# Autodesk Inventor assembly: Right Rear Wheel with hub
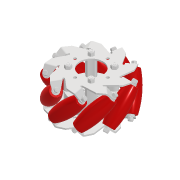
[picture p0: Inventor's stored thumbnail of the model, 180x180]
Saved by Autodesk Inventor 2020 (Build 240168000, 168)
## iProperties
Created: 2020-02-22
Part Number: Right Rear Wheel with hub
Document SubType Name: Assembly
Designer: ball
Author: ball
## Documents named in this file (5)
- C:\FTC\FTC8863CAD\2019 Robot\Mecanum Drive Train Metal\Right Rear Wheel with hub.iam
- C:\FTC\FTC8863CAD\GoBilda\1310 Parts\1310-0016-4008 assembly.ipt
- C:\FTC\FTC8863CAD\StepLibraries\Screws\M4 x 22 SOCKET HEAD CAP SCREW.ipt
- C:\FTC\FTC8863CAD\StepLibraries\Washers\M4 FLAT WASHER.ipt
- C:\FTC\FTC8863CAD\GoBilda\3213 Parts\3606-0000-0100 assembly.iam
## Components (10 placed, 4 different names)
1. 3606-0000-0100 assembly:1 [sub-assembly] — Mate:1, Mate:2, Mate:3, Mate:12, Mate:13, Mate:14, Mate:15, Mate:18, Mate:19, Mate:22, Mate:23
2. 1310-0016-4008 assembly:1 — Mate:1, Mate:2, Mate:3
3. M4 x 22 SOCKET HEAD CAP SCREW:1 — Mate:13
4. M4 FLAT WASHER:1 — Mate:12
5. M4 x 22 SOCKET HEAD CAP SCREW:3 — Mate:19
6. M4 FLAT WASHER:3 — Mate:18
7. M4 x 22 SOCKET HEAD CAP SCREW:4 — Mate:15
8. M4 FLAT WASHER:4 — Mate:14
9. M4 x 22 SOCKET HEAD CAP SCREW:5 — Mate:23
10. M4 FLAT WASHER:5 — Mate:22
## Relationships (19: Mate 19)
- Mate:1: 3606-0000-0100 assembly:1 ↔ 1310-0016-4008 assembly:1
- Mate:2: 3606-0000-0100 assembly:1 ↔ 1310-0016-4008 assembly:1
- Mate:3: 3606-0000-0100 assembly:1 ↔ 1310-0016-4008 assembly:1
- [Mate]: M4 x 22 SOCKET HEAD CAP SCREW:1 ↔ M4 FLAT WASHER:1
- [Mate]: M4 x 22 SOCKET HEAD CAP SCREW:1 ↔ M4 FLAT WASHER:1
- [Mate]: M4 x 22 SOCKET HEAD CAP SCREW:3 ↔ M4 FLAT WASHER:3
- [Mate]: M4 x 22 SOCKET HEAD CAP SCREW:3 ↔ M4 FLAT WASHER:3
- [Mate]: M4 x 22 SOCKET HEAD CAP SCREW:4 ↔ M4 FLAT WASHER:4
- [Mate]: M4 x 22 SOCKET HEAD CAP SCREW:4 ↔ M4 FLAT WASHER:4
- Mate:12: 3606-0000-0100 assembly:1 ↔ M4 FLAT WASHER:1
- Mate:13: 3606-0000-0100 assembly:1 ↔ M4 x 22 SOCKET HEAD CAP SCREW:1
- Mate:14: 3606-0000-0100 assembly:1 ↔ M4 FLAT WASHER:4
- Mate:15: 3606-0000-0100 assembly:1 ↔ M4 x 22 SOCKET HEAD CAP SCREW:4
- Mate:18: 3606-0000-0100 assembly:1 ↔ M4 FLAT WASHER:3
- Mate:19: 3606-0000-0100 assembly:1 ↔ M4 x 22 SOCKET HEAD CAP SCREW:3
- [Mate]: M4 x 22 SOCKET HEAD CAP SCREW:5 ↔ M4 FLAT WASHER:5
- [Mate]: M4 x 22 SOCKET HEAD CAP SCREW:5 ↔ M4 FLAT WASHER:5
- Mate:22: 3606-0000-0100 assembly:1 ↔ M4 FLAT WASHER:5
- Mate:23: 3606-0000-0100 assembly:1 ↔ M4 x 22 SOCKET HEAD CAP SCREW:5
## Named parameters: d14_d12 = 0 mm, d15_d13 = 0 mm, d37_d14_d12 = 0 mm, d38_d15_d13 = 0 mm, d39_d14_d12 = 0 mm, d40_d15_d13 = 0 mm, d49_d14_d12 = 0 mm, d50_d15_d13 = 0 mm
